# Autodesk Inventor assembly: Slider Crank
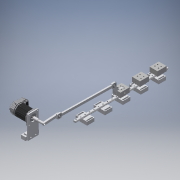
[picture p0: Inventor's stored thumbnail of the model, 180x180]
Saved by Autodesk Inventor 2016 (Build 200138000, 138)
## iProperties
Created: 2015-06-08
Part Number: Slider Crank
Document SubType Name: Assembly
Designer: Dennis
Author: Dennis
## Documents named in this file (7)
- C:\Users\Dennis\Dropbox\NI Work\NI Slider Crank\Slider Crank - FINAL.iam
- C:\Users\Dennis\Dropbox\NI Work\NI Slider Crank\Assemblies\Fixed Parts.iam
- C:\Users\Dennis\Dropbox\NI Work\NI Slider Crank\Assemblies\Long Arm.iam
- C:\Users\Dennis\Dropbox\NI Work\NI Slider Crank\Assemblies\Mass 1.iam
- C:\Users\Dennis\Dropbox\NI Work\NI Slider Crank\Assemblies\Mass 2.iam
- C:\Users\Dennis\Dropbox\NI Work\NI Slider Crank\Assemblies\Mass 3.iam
- C:\Users\Dennis\Dropbox\NI Work\NI Slider Crank\Assemblies\Short Arm.iam
## Components (6 placed, 6 different names)
1. Fixed Parts:1 [sub-assembly] — Mate:1, Mate:4, Mate:5, Mate:6, Mate:7, Mate:8, Mate:9
2. Long Arm:1 [sub-assembly] — Mate:2, Mate:3, Mate:10, Mate:11
3. Mass 1:1 [sub-assembly] — Mate:4, Mate:5, Mate:10, Mate:11
4. Mass 2:1 [sub-assembly] — Mate:6, Mate:7
5. Mass 3:1 [sub-assembly] — Mate:8, Mate:9
6. Short Arm:1 [sub-assembly] — Mate:1, Mate:2, Mate:3
## Relationships (11: Mate 11)
- Mate:1: Fixed Parts:1 ↔ Short Arm:1
- Mate:2: Long Arm:1 ↔ Short Arm:1
- Mate:3: Long Arm:1 ↔ Short Arm:1
- Mate:4: Fixed Parts:1 ↔ Mass 1:1
- Mate:5: Fixed Parts:1 ↔ Mass 1:1
- Mate:6: Fixed Parts:1 ↔ Mass 2:1
- Mate:7: Fixed Parts:1 ↔ Mass 2:1
- Mate:8: Fixed Parts:1 ↔ Mass 3:1
- Mate:9: Fixed Parts:1 ↔ Mass 3:1
- Mate:10: Long Arm:1 ↔ Mass 1:1
- Mate:11: Long Arm:1 ↔ Mass 1:1
